# Autodesk Inventor assembly: modified
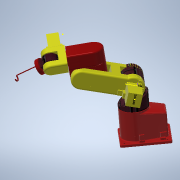
[picture p0: Inventor's stored thumbnail of the model, 180x180]
Saved by Autodesk Inventor 2021 (Build 250183000, 183)
## iProperties
Created: 2015-10-07
Part Number: modified
Document SubType Name: Assembly
Designer: 1348487
Author: 1348487
## Documents named in this file (9)
- C:\Users\HP\Downloads\modified.iam
- C:\Users\HP\Documents\handling unit\Robot-Base-Model-A.ipt
- C:\Users\HP\Downloads\Robot-Axis1-2.ipt
- C:\Users\HP\Downloads\Robot-Axis2-3.ipt
- C:\Users\HP\Downloads\Robot-Axis3-4.ipt
- C:\Users\HP\Documents\handling unit\Robot-Axis4-5.ipt
- C:\Users\HP\Downloads\Robot-Axis5.ipt
- C:\Users\HP\Downloads\Robot-Axis5-Adapter.ipt
- U:\Documents\inventor_drafting\Robot-GripperAssy.iam
## Components (8 placed, 8 different names)
1. Robot-Base-Model-A:1 — Mate:1, Mate:2, Angle:1
2. Robot-Axis1-2:1 — Mate:1, Mate:2, Angle:1, Mate:3, Mate:4, Flush:1, Flush:2, Flush:3
3. Robot-Axis2-3:1 — Mate:3, Mate:4, Mate:7, Mate:6, Angle:2, Flush:1, Flush:2, Flush:3
4. Robot-Axis3-4:1 — Mate:7, Mate:6, Angle:2, Insert:1
5. Robot-Axis4-5:1 — Insert:1, Mate:8, Mate:9
6. Robot-Axis5:1 — Insert:2, Mate:8, Mate:9
7. Robot-Axis5-Adapter:1 — Insert:2, Mate:10, Mate:11, Mate:12
8. Robot-GripperAssy:1 [sub-assembly] — Mate:10, Mate:11, Mate:12
## Relationships (18: Mate 11, Flush 3, Angle 2, Insert 2)
- Mate:1: Robot-Base-Model-A:1 ↔ Robot-Axis1-2:1
- Mate:2: Robot-Base-Model-A:1 ↔ Robot-Axis1-2:1
- Angle:1 (0 deg): Robot-Base-Model-A:1 ↔ Robot-Axis1-2:1
- Mate:3: Robot-Axis1-2:1 ↔ Robot-Axis2-3:1
- Mate:4: Robot-Axis1-2:1 ↔ Robot-Axis2-3:1
- Mate:7: Robot-Axis2-3:1 ↔ Robot-Axis3-4:1
- Mate:6: Robot-Axis2-3:1 ↔ Robot-Axis3-4:1
- Angle:2 (20 deg): Robot-Axis2-3:1 ↔ Robot-Axis3-4:1
- Insert:1: Robot-Axis3-4:1 ↔ Robot-Axis4-5:1
- Insert:2: Robot-Axis5:1 ↔ Robot-Axis5-Adapter:1
- Mate:8: Robot-Axis4-5:1 ↔ Robot-Axis5:1
- Mate:9: Robot-Axis4-5:1 ↔ Robot-Axis5:1
- Mate:10: Robot-Axis5-Adapter:1 ↔ Robot-GripperAssy:1
- Mate:11: Robot-Axis5-Adapter:1 ↔ Robot-GripperAssy:1
- Mate:12: Robot-Axis5-Adapter:1 ↔ Robot-GripperAssy:1
- Flush:1: Robot-Axis1-2:1 ↔ Robot-Axis2-3:1
- Flush:2: Robot-Axis1-2:1 ↔ Robot-Axis2-3:1
- Flush:3: Robot-Axis1-2:1 ↔ Robot-Axis2-3:1
